# Autodesk Inventor assembly: Slider-Crank_JacobMorgan_040915_pd3
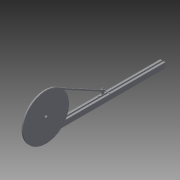
[picture p0: Inventor's stored thumbnail of the model, 180x180]
Saved by Autodesk Inventor 2015 (Build 190159000, 159)
## iProperties
Created: 2015-04-09
Part Number: Slider-Crank_JacobMorgan_040915_pd3
Document SubType Name: Assembly
Designer: WASHHSST
Author: WASHHSST
## Documents named in this file (8)
- C:\Users\washhsst\Documents\GitHub\myWork\Slider-Crank\Slider-Crank_JacobMorgan_040915_pd3.iam
- C:\Users\washhsst\Documents\GitHub\myWork\Slider-Crank\rail.ipt
- C:\Users\washhsst\Documents\GitHub\myWork\Slider-Crank\slider.ipt
- C:\Users\washhsst\Documents\GitHub\myWork\Slider-Crank\rotator.ipt
- C:\Users\washhsst\Documents\GitHub\myWork\Slider-Crank\rotator_Base.ipt
- C:\Users\washhsst\Documents\GitHub\myWork\Slider-Crank\sliderArmPin.ipt
- C:\Users\washhsst\Documents\GitHub\myWork\Slider-Crank\long_Pin.ipt
- C:\Users\washhsst\Documents\GitHub\myWork\Slider-Crank\rod.ipt
## Components (7 placed, 7 different names)
1. rail:1 — Mate:1, Mate:2, Mate:3, Mate:4, Mate:5
2. slider:1 — Mate:1, Mate:2, Mate:11, Mate:12, Mate:13
3. rotator:1 — Mate:7, Insert:1, Mate:8, Mate:10
4. rotator_Base:1 — Mate:3, Mate:4, Mate:5, Mate:7, Mate:8, Mate:12
5. sliderArmPin:1 — Insert:1, Mate:9
6. long_Pin:1 — Mate:11, Mate:13, Mate:14
7. rod:1 — Mate:9, Mate:10, Mate:14
## Relationships (14: Mate 13, Insert 1)
- Mate:1: rail:1 ↔ slider:1
- Mate:2: rail:1 ↔ slider:1
- Mate:3: rail:1 ↔ rotator_Base:1
- Mate:4: rail:1 ↔ rotator_Base:1
- Mate:5: rail:1 ↔ rotator_Base:1
- Mate:7: rotator:1 ↔ rotator_Base:1
- Insert:1: rotator:1 ↔ sliderArmPin:1
- Mate:8: rotator:1 ↔ rotator_Base:1
- Mate:9: sliderArmPin:1 ↔ rod:1
- Mate:10: rotator:1 ↔ rod:1
- Mate:11: slider:1 ↔ long_Pin:1
- Mate:12: slider:1 ↔ rotator_Base:1
- Mate:13: slider:1 ↔ long_Pin:1
- Mate:14: long_Pin:1 ↔ rod:1
